# Autodesk Inventor assembly: Vented plug
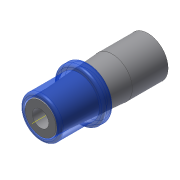
[picture p0: Inventor's stored thumbnail of the model, 180x180]
Saved by Autodesk Inventor 2014 (Build 180170000, 170)
## iProperties
Created: 2016-08-28
Part Number: Vented plug
Document SubType Name: Assembly
Designer: Camilo
Author: Camilo
## Documents named in this file (3)
- Z:\Github\AgingTests\3D parts\Vented plug\Vented plug.iam
- Z:\Github\AgingTests\3D parts\ECoG holder\flaskPort.ipt
- Z:\Github\AgingTests\3D parts\Vented plug\Vented_plug.ipt
## Components (2 placed, 2 different names)
1. flaskPort:1 — Mate:1, Flush:1, Mate:2, Flush:2
2. Vented_plug:1 — Flush:2
## Relationships (4: Mate 2, Flush 2)
- Mate:1: flaskPort:1
- Flush:1: flaskPort:1
- Mate:2: flaskPort:1
- Flush:2: flaskPort:1 ↔ Vented_plug:1
